# Autodesk Inventor assembly: 000.003 - Блок АКБ СБ
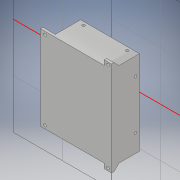
[picture p0: Inventor's stored thumbnail of the model, 180x180]
Saved by Autodesk Inventor 2022 (Build 260153000, 153)
## iProperties
Created: 2022-02-26
Part Number: 000.003 - Блок АКБ СБ
Document SubType Name: Assembly
Designer: Petrov Ivan
Author: Petrov Ivan
## Documents named in this file (3)
- D:\IVAN\Ivan_desktop\Kvantorium\Projects\YouBotRobot\design\000.003 - Блок АКБ СБ.iam
- D:\IVAN\Ivan_desktop\Kvantorium\Projects\YouBotRobot\design\000.003.001 - Основание.ipt
- D:\IVAN\Ivan_desktop\Kvantorium\Projects\YouBotRobot\design\standart_components\NUCLEO.ipt
## Components (3 placed, 2 different names)
1. 000.003.001 - Основание:1 — Совмещение:5, Совмещение:6, Совмещение:7
2. NUCLEO:3 — Совмещение:6, Заподлицо:2
3. NUCLEO:4 — Совмещение:5, Совмещение:7, Заподлицо:2
## Relationships (4: Mate 3, Flush 1)
- Совмещение:5 [Mate]: 000.003.001 - Основание:1 ↔ NUCLEO:4
- Совмещение:6 [Mate]: 000.003.001 - Основание:1 ↔ NUCLEO:3
- Совмещение:7 [Mate] (18 mm): 000.003.001 - Основание:1 ↔ NUCLEO:4
- Заподлицо:2 [Flush]: NUCLEO:3 ↔ NUCLEO:4
